# Autodesk Inventor assembly: CLS24.5
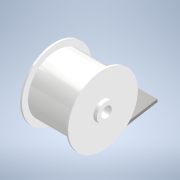
[picture p0: Inventor's stored thumbnail of the model, 180x180]
Saved by Autodesk Inventor 2021 (Build 250183000, 183)
## iProperties
Created: 2021-01-01
Part Number: CLS24.5
Document SubType Name: Assembly
Designer: YusukeKunita
Author: YusukeKunita
## Documents named in this file (3)
- C:\Users\YusukeKunita\Documents\GrabCAD\NHK2021\BasicParts\よく使う部品（萩原）\ConstantLoadSpring\CLS_24.5N\CLS_24.5N.iam
- C:\Users\YusukeKunita\Documents\GrabCAD\NHK2021\BasicParts\よく使う部品（萩原）\ConstantLoadSpring\CLS_24.5N\CLS_24.5N.ipt
- C:\Users\YusukeKunita\Documents\GrabCAD\NHK2021\BasicParts\よく使う部品（萩原）\ConstantLoadSpring\CLS_24.5N\CLS_24.5N_plate.ipt
## Components (2 placed, 2 different names)
1. CLS_24.5N:1 — 正接:1, 正接:2, メイト:1
2. CLS_24.5N_plate:1 — 正接:1, 正接:2, メイト:1
## Relationships (3: Tangent 2, Mate 1)
- 正接:1 [Tangent]: CLS_24.5N:1 ↔ CLS_24.5N_plate:1
- 正接:2 [Tangent]: CLS_24.5N:1 ↔ CLS_24.5N_plate:1
- メイト:1 [Mate] (0.25 mm): CLS_24.5N:1 ↔ CLS_24.5N_plate:1
